# Autodesk Inventor assembly: RT_ARM_A_003
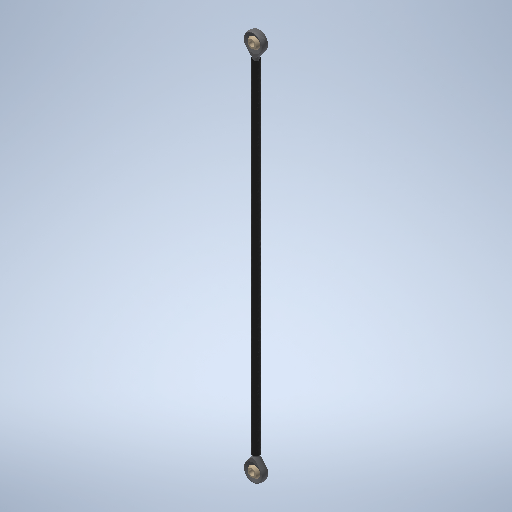
[picture p0: Inventor's stored thumbnail of the model, 512x512]
Saved by Autodesk Inventor 2025.3 (Build 293356000, 356)
## iProperties
Created: 2026-05-13
Part Number: RT_ARM_A_003
Document SubType Name: Assembly
Designer: louis
Author: louis
## Documents named in this file (3)
- C:\Users\louis\OneDrive\Desktop\R_Trident\02_CAD\04_Subassemblies\RT_ARM_A_003.iam
- C:\Users\louis\OneDrive\Desktop\R_Trident\02_CAD\03_Parts_Custom\RT_ARM_MC_006_Forearm.ipt
- C:\Users\louis\OneDrive\Desktop\R_Trident\02_CAD\01_Standard_Parts\KALM_05_CL_1\KALM_05_CL_1\KALM_05_CL_1.iam
## Components (3 placed, 2 different names)
1. RT_ARM_MC_006_Forearm:1 — Mate:1, Mate:2, Mate:3, Mate:4, Mate:5, Mate:6, Mate:7
2. KALM_05_CL_1:1 [sub-assembly] — Mate:4, Mate:7, Flush:10
3. KALM_05_CL_1:2 [sub-assembly] — Mate:5, Mate:6, Mate:8, Flush:10
## Relationships (9: Mate 8, Flush 1)
- Mate:1: RT_ARM_MC_006_Forearm:1
- Mate:2: RT_ARM_MC_006_Forearm:1
- Mate:3: RT_ARM_MC_006_Forearm:1
- Mate:4: RT_ARM_MC_006_Forearm:1 ↔ KALM_05_CL_1:1
- Mate:5: RT_ARM_MC_006_Forearm:1 ↔ KALM_05_CL_1:2
- Mate:6 (14 mm): RT_ARM_MC_006_Forearm:1 ↔ KALM_05_CL_1:2
- Mate:7 (14 mm): RT_ARM_MC_006_Forearm:1 ↔ KALM_05_CL_1:1
- Mate:8: KALM_05_CL_1:2
- Flush:10: KALM_05_CL_1:1 ↔ KALM_05_CL_1:2
